# Autodesk Inventor assembly: carriage
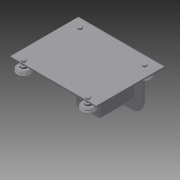
[picture p0: Inventor's stored thumbnail of the model, 180x180]
Saved by Autodesk Inventor 2013 (Build 170138000, 138)
## iProperties
Created: 2012-12-03
Part Number: carriage
Document SubType Name: Assembly
Designer: Istvan
Author: Istvan
## Documents named in this file (4)
- D:\GitHub\Crown-Fire\CAD\Frame\y-carriage\carriage.iam
- D:\GitHub\Crown-Fire\CAD\Frame\y-carriage\backplate.ipt
- D:\GitHub\Crown-Fire\CAD\Hardware\Bearings\DualVee-size2.ipt
- D:\GitHub\Crown-Fire\CAD\Electronics\Motors\G723-280-4.ipt
## Components (6 placed, 3 different names)
1. backplate:1 — Mate:1, Mate:2, Mate:3, Mate:4, Mate:5, Mate:6
2. DualVee-size2:1 — Mate:3, Flush:1, Flush:2, Flush:3
3. DualVee-size2:2 — Mate:4, Flush:1
4. DualVee-size2:3 — Mate:2, Flush:3
5. DualVee-size2:4 — Mate:1, Flush:2
6. G723-280-4:1 — Mate:5, Mate:6
## Relationships (9: Mate 6, Flush 3)
- Mate:1: backplate:1 ↔ DualVee-size2:4
- Mate:2: backplate:1 ↔ DualVee-size2:3
- Mate:3: backplate:1 ↔ DualVee-size2:1
- Mate:4: backplate:1 ↔ DualVee-size2:2
- Flush:1: DualVee-size2:1 ↔ DualVee-size2:2
- Flush:2: DualVee-size2:1 ↔ DualVee-size2:4
- Flush:3: DualVee-size2:1 ↔ DualVee-size2:3
- Mate:5: backplate:1 ↔ G723-280-4:1
- Mate:6: backplate:1 ↔ G723-280-4:1
